# Autodesk Inventor assembly: 61581400
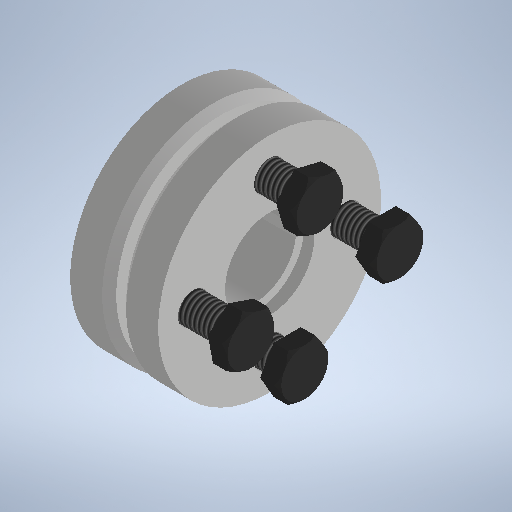
[picture p0: Inventor's stored thumbnail of the model, 512x512]
Saved by Autodesk Inventor 2025.4 (Build 294407000, 407)
## iProperties
Category: PARTsolutions
Company: MAEDLER
Created: 2026-05-06
Part Number: 61581400
Catalog Web Link: www.3dfindit.com
Description: MAE-SCHRSCHEI-ST-Shrink Disks ST, For very high torques
Vendor: MAEDLER
Document SubType Name: Assembly
Designer: psAdmin
Manufacturer: MAEDLER
Mass: 100 g
Surface Area: 89.6051 cm^2
Volume: 13.5691 cm^3
Density: 7.3697 g/cm^3
PSOL_IDENT_0: {$CADENAS_DATA/23d-libs/maedler/antriebselemente/spannbuchsen_und_spannsaetze/schrumpfscheiben/schru
PSOL_IDENT_1: mpfscheibe_st/schrumpfscheibe_st.prj},180 {VTYP=3D},{STYP=ASSTAB},{NB=61581400},{LINA=61581400},{NN=
PSOL_IDENT_2: MAE-SCHRSCHEI-ST},{DATE=10.03.2025 09:23:18},{GEOMDATE=02.01.2025 14:54:34},{VERSION=},{LINEID=20},{
PSOL_IDENT_3: WBVAR=},{WBNUMERIC=}  {NB=61581400},{LINA=61581400},{KT=DUMMY},{ARTNR=61581400},{WEBSHOP=Produktdeta
PSOL_IDENT_4: ils / Katalogseite / Montageanleitung},{MATK=Stahl},{MAT=Hochwertiger Stahl 42CrMo4},{ID=14},{DW=10
PSOL_IDENT_5: / 11 / 12},{DM=40 / 50 / 65},{D=38},{L=15.0},{L2=18.5},{I=10},{E=2.50},{PSMAX=0.014},{SCHR= 4 x M5 x
PSOL_IDENT_6: 12},{TA=3},{PW=154 / 191 / 243},{GEW=0.10},{TK=26.0},{SSA=4},{SSG=5},{SSL=12},{K=3.5},{SDW=6.9},{SW=
PSOL_IDENT_7: 8},{HDW=0.5},{DG=5.3},{D1L=20.00},{D2L=16.80},{SL=1.70},{HD=35.6},{BA=6.650},{TN=dummy_schrschei_st_
PSOL_IDENT_8: 14},{CTN=84839089},{DIST=1.883333},{PPATH=schrschei_st_sbl.prj},{CNSDWTEMPLATE=_dw/ansicht_right_fro
PSOL_IDENT_9: nt.dw}
NB: 61581400
NN: MAE-SCHRSCHEI-ST
NT: Shrink Disks ST, For very high torques
NBSYN: $ARTNR.
LINA: 61581400
CATALOG: MÄDLER
ARTNR: 61581400
WEBSHOP: Product details / Catalogue page / Assembly instructions
MATK: Steel
MAT: High-quality steel 42CrMo4
ID: 14
DW: 10 / 11 / 12
DM: 40 / 50 / 65
D: 38
L: 15
L2: 18.5
I: 10
E: 2.5
PSMAX: 0.014
SCHR: 4 x M5 x 12
TA: 3
PW: 154 / 191 / 243
GEW: 0.1
CTN: 84839089
SUPPLIER: MAEDLER
ARTICLENO: 61581400
BOMINFO: 61581400
CREATOR: CADENAS GmbH
Title: 61581400
Author: Cadenas PARTsolutions
Comments: Shrink Disks ST, For very high torques
## Documents named in this file (5)
- C:\Users\louis\OneDrive\Desktop\R_Trident\02_CAD\01_Standard_Parts\615 814 00\61581400.iam
- C:\Users\louis\OneDrive\Desktop\R_Trident\02_CAD\01_Standard_Parts\615 814 00\61581400_2.ipt
- C:\Users\louis\OneDrive\Desktop\R_Trident\02_CAD\01_Standard_Parts\615 814 00\61581400_3.ipt
- C:\Users\louis\OneDrive\Desktop\R_Trident\02_CAD\01_Standard_Parts\615 814 00\61581400_4.ipt
- C:\Users\louis\OneDrive\Desktop\R_Trident\02_CAD\01_Standard_Parts\615 814 00\61581400_5.ipt
## Components (7 placed, 4 different names)
1. 61581400_2:1
2. 61581400_3:1
3. 61581400_4:1 — Mate:1, Mate:2, Mate:3, Mate:4
4. 61581400_5:1 — Mate:4
5. 61581400_5:2 — Mate:3
6. 61581400_5:3 — Mate:2
7. 61581400_5:4 — Mate:1
## Relationships (4: Mate 4)
- Mate:1: 61581400_4:1 ↔ 61581400_5:4
- Mate:2: 61581400_4:1 ↔ 61581400_5:3
- Mate:3: 61581400_4:1 ↔ 61581400_5:2
- Mate:4: 61581400_4:1 ↔ 61581400_5:1
